# Autodesk Inventor assembly: 사각형 OV-PAM 5패턴
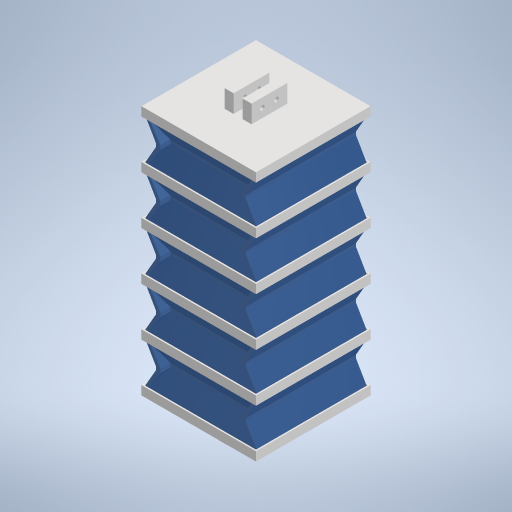
[picture p0: Inventor's stored thumbnail of the model, 512x512]
Saved by Autodesk Inventor 2024 (Build 280153000, 153)
## iProperties
Created: 2023-06-16
Part Number: 사각형 OV-PAM 5패턴
Document SubType Name: Assembly
Designer: jsw
Author: jsw
## Documents named in this file (5)
- C:\승원\co-op\OV-PAM\square OV-PAM 5 patterns.iam
- C:\승원\co-op\OV-PAM\사각형 OV-PAM 5패턴 층 한개.ipt
- C:\승원\co-op\OV-PAM\사각형 OV-PAM 5패턴 상단.ipt
- C:\승원\co-op\OV-PAM\사각형 OV-PAM 5패턴 하단.ipt
- C:\승원\co-op\OV-PAM\사각형 OV-PAM 5패턴 링.ipt
## Components (11 placed, 4 different names)
1. 사각형 OV-PAM 5패턴 상단:1 — 메이트:1, 메이트:2, 메이트:3
2. 사각형 OV-PAM 5패턴 층 한개:5 — 메이트:7, 메이트:8, 메이트:9, 메이트:10, 메이트:11, 메이트:12
3. 사각형 OV-PAM 5패턴 하단:1 — 메이트:10, 메이트:11, 메이트:12
4. 사각형 OV-PAM 5패턴 층 한개:1 — 메이트:1, 메이트:2, 메이트:3, 메이트:4, 메이트:5, 메이트:6
5. 사각형 OV-PAM 5패턴 링:1 — 메이트:4, 메이트:5, 메이트:6
6. 사각형 OV-PAM 5패턴 층 한개:2
7. 사각형 OV-PAM 5패턴 링:2
8. 사각형 OV-PAM 5패턴 층 한개:3
9. 사각형 OV-PAM 5패턴 링:3
10. 사각형 OV-PAM 5패턴 층 한개:4
11. 사각형 OV-PAM 5패턴 링:4 — 메이트:7, 메이트:8, 메이트:9
## Component patterns: (4 elements, first: 사각형 OV-PAM 5패턴 층 한개:1 + 사각형 OV-PAM 5패턴 링:1)
## Relationships (12: Mate 12)
- 메이트:1 [Mate]: 사각형 OV-PAM 5패턴 상단:1 ↔ 사각형 OV-PAM 5패턴 층 한개:1
- 메이트:2 [Mate]: 사각형 OV-PAM 5패턴 상단:1 ↔ 사각형 OV-PAM 5패턴 층 한개:1
- 메이트:3 [Mate]: 사각형 OV-PAM 5패턴 상단:1 ↔ 사각형 OV-PAM 5패턴 층 한개:1
- 메이트:4 [Mate]: 사각형 OV-PAM 5패턴 층 한개:1 ↔ 사각형 OV-PAM 5패턴 링:1
- 메이트:5 [Mate]: 사각형 OV-PAM 5패턴 층 한개:1 ↔ 사각형 OV-PAM 5패턴 링:1
- 메이트:6 [Mate]: 사각형 OV-PAM 5패턴 층 한개:1 ↔ 사각형 OV-PAM 5패턴 링:1
- 메이트:7 [Mate]: 사각형 OV-PAM 5패턴 층 한개:5 ↔ 사각형 OV-PAM 5패턴 링:4
- 메이트:8 [Mate]: 사각형 OV-PAM 5패턴 층 한개:5 ↔ 사각형 OV-PAM 5패턴 링:4
- 메이트:9 [Mate]: 사각형 OV-PAM 5패턴 층 한개:5 ↔ 사각형 OV-PAM 5패턴 링:4
- 메이트:10 [Mate]: 사각형 OV-PAM 5패턴 층 한개:5 ↔ 사각형 OV-PAM 5패턴 하단:1
- 메이트:11 [Mate]: 사각형 OV-PAM 5패턴 층 한개:5 ↔ 사각형 OV-PAM 5패턴 하단:1
- 메이트:12 [Mate]: 사각형 OV-PAM 5패턴 층 한개:5 ↔ 사각형 OV-PAM 5패턴 하단:1
